# Autodesk Inventor assembly: pcb_stack_tall
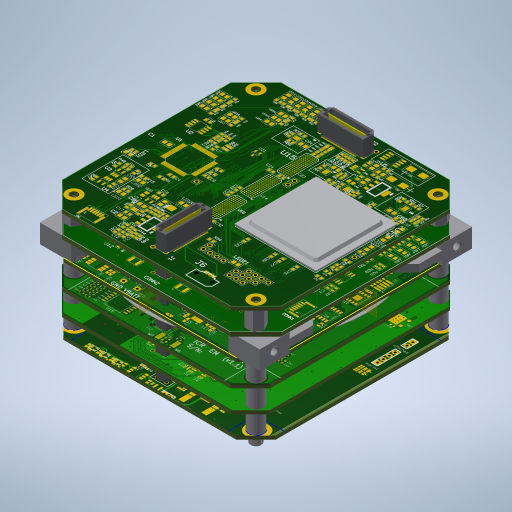
[picture p0: Inventor's stored thumbnail of the model, 512x512]
Saved by Autodesk Inventor 2023 (Build 270158000, 158)
## iProperties
Created: 2018-06-10
Part Number: pcb_stack_tall
Document SubType Name: Assembly
Designer: RDavis
Author: RDavis
## Documents named in this file (11)
- E:\Dropbox\AMSAT\CAD_backup_frequent_files_20200629\pcb_stack_tall.iam
- E:\Dropbox\AMSAT\CAD_backup_frequent_files_20200629\PCB_VUC.iam
- E:\Dropbox\AMSAT\CAD_backup_frequent_files_20200629\standoff815mm.ipt
- E:\Dropbox\AMSAT\CAD_backup_frequent_files_20200629\PCB_LEPF.iam
- E:\Dropbox\AMSAT\CAD_backup_frequent_files_20200629\PCB_RT-IHU.iam
- E:\Dropbox\AMSAT\CAD_backup_frequent_files_20200629\PCB_LT_RX-TX.iam
- E:\Dropbox\AMSAT\CAD_backup_frequent_files_20200629\PCB_LT_ICR.iam
- E:\Dropbox\AMSAT\CAD_backup_frequent_files_20200629\NAS620-4L.ipt
- E:\Dropbox\AMSAT\CAD_backup_frequent_files_20200629\PCB_LIHU.iam
- E:\Dropbox\AMSAT\CAD_backup_frequent_files_20200629\spacer_threaded.ipt
- E:\Dropbox\AMSAT\CAD_backup_frequent_files_20200629\Imported Components\92185A128_shcs_4-40_1_75\92185A128_shcs_4-40_1_75.ipt
## Components (30 placed, 10 different names)
1. PCB_LIHU:1 [sub-assembly] — Insert:6, Insert:7, Insert:8, Insert:9, Angle:6, Insert:58, Insert:59, Insert:60, Insert:61
2. standoff815mm:17 — Insert:6, Insert:14
3. standoff815mm:18 — Insert:7
4. standoff815mm:19 — Insert:8
5. standoff815mm:20 — Insert:9
6. PCB_LT_RX-TX:1 [sub-assembly] — Insert:14, Angle:6, Insert:15, Insert:16, Insert:17, Insert:18, Angle:7, Insert:57
7. standoff815mm:5 — Insert:15, Insert:19, Insert:56, Insert:57
8. standoff815mm:6 — Insert:16
9. standoff815mm:7 — Insert:17
10. standoff815mm:8 — Insert:18
11. PCB_LT_ICR:1 [sub-assembly] — Insert:19, Angle:7, Insert:20, Insert:21, Insert:22, Insert:23, Angle:8, Insert:56
12. standoff815mm:9 — Insert:20
13. standoff815mm:10 — Insert:21
14. standoff815mm:11 — Insert:22
15. standoff815mm:12 — Insert:23
16. PCB_RT-IHU:1 [sub-assembly] — Angle:8, Angle:13, Insert:55
17. PCB_VUC:1 [sub-assembly] — Angle:13, Angle:14, Insert:55, Insert:62, Insert:63, Insert:64, Insert:65
18. spacer_threaded:1 — Insert:62
19. spacer_threaded:2 — Insert:63
20. spacer_threaded:3 — Insert:64
21. spacer_threaded:4 — Insert:65
22. PCB_LEPF:1 [sub-assembly] — Angle:14
23. NAS620-4L:1 — Insert:60, Insert:67
24. NAS620-4L:2 — Insert:61, Insert:66
25. NAS620-4L:3 — Insert:58, Insert:69
26. NAS620-4L:4 — Insert:59, Insert:68
27. 92185A128_shcs_4-40_1_75:1 — Insert:66
28. 92185A128_shcs_4-40_1_75:2 — Insert:67
29. 92185A128_shcs_4-40_1_75:3 — Insert:68
30. 92185A128_shcs_4-40_1_75:4 — Insert:69
## Relationships (34: Insert 29, Angle 5)
- Insert:6: PCB_LIHU:1 ↔ standoff815mm:17
- Insert:7: PCB_LIHU:1 ↔ standoff815mm:18
- Insert:8: PCB_LIHU:1 ↔ standoff815mm:19
- Insert:9: PCB_LIHU:1 ↔ standoff815mm:20
- Insert:14: standoff815mm:17 ↔ PCB_LT_RX-TX:1
- Angle:6 (0 deg): PCB_LIHU:1 ↔ PCB_LT_RX-TX:1
- Insert:15: PCB_LT_RX-TX:1 ↔ standoff815mm:5
- Insert:16: PCB_LT_RX-TX:1 ↔ standoff815mm:6
- Insert:17: PCB_LT_RX-TX:1 ↔ standoff815mm:7
- Insert:18: PCB_LT_RX-TX:1 ↔ standoff815mm:8
- Insert:19: standoff815mm:5 ↔ PCB_LT_ICR:1
- Angle:7 (0 deg): PCB_LT_RX-TX:1 ↔ PCB_LT_ICR:1
- Insert:20: PCB_LT_ICR:1 ↔ standoff815mm:9
- Insert:21: PCB_LT_ICR:1 ↔ standoff815mm:10
- Insert:22: PCB_LT_ICR:1 ↔ standoff815mm:11
- Insert:23: PCB_LT_ICR:1 ↔ standoff815mm:12
- Angle:8 (0 deg): PCB_LT_ICR:1 ↔ PCB_RT-IHU:1
- Angle:13 (0 deg): PCB_RT-IHU:1 ↔ PCB_VUC:1
- Angle:14 (0 deg): PCB_VUC:1 ↔ PCB_LEPF:1
- Insert:55: PCB_RT-IHU:1 ↔ PCB_VUC:1
- Insert:56: standoff815mm:5 ↔ PCB_LT_ICR:1
- Insert:57: PCB_LT_RX-TX:1 ↔ standoff815mm:5
- Insert:58: PCB_LIHU:1 ↔ NAS620-4L:3
- Insert:59: PCB_LIHU:1 ↔ NAS620-4L:4
- Insert:60: PCB_LIHU:1 ↔ NAS620-4L:1
- Insert:61: PCB_LIHU:1 ↔ NAS620-4L:2
- Insert:62: PCB_VUC:1 ↔ spacer_threaded:1
- Insert:63: PCB_VUC:1 ↔ spacer_threaded:2
- Insert:64: PCB_VUC:1 ↔ spacer_threaded:3
- Insert:65: PCB_VUC:1 ↔ spacer_threaded:4
- Insert:66: NAS620-4L:2 ↔ 92185A128_shcs_4-40_1_75:1
- Insert:67: NAS620-4L:1 ↔ 92185A128_shcs_4-40_1_75:2
- Insert:68: NAS620-4L:4 ↔ 92185A128_shcs_4-40_1_75:3
- Insert:69: NAS620-4L:3 ↔ 92185A128_shcs_4-40_1_75:4
